# Autodesk Inventor assembly: ASY MSC 200 BACK
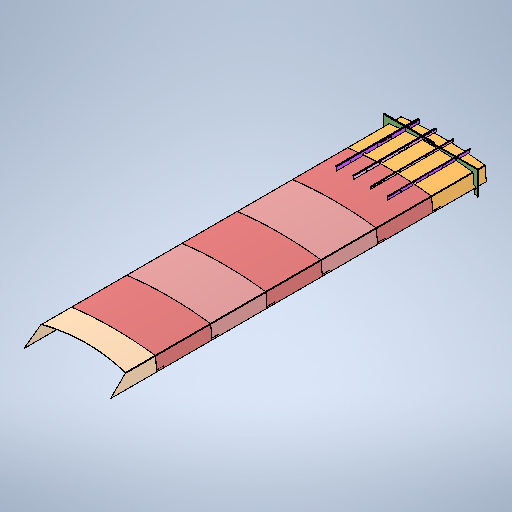
[picture p0: Inventor's stored thumbnail of the model, 512x512]
Saved by Autodesk Inventor 2025 (Build 290162010, 162A)
## iProperties
Created: 2024-07-19
Part Number: ASY MSC 200 BACK
Document SubType Name: Assembly
Designer: pokla
Stock Number: ASY МОО 200 спина
Mass: 379257 g
Surface Area: 351509 cm^2
Volume: 47407.1 cm^3
Density: 8 g/cm^3
Author: pokla
## Documents named in this file (10)
- C:\Users\admin\YandexDisk-badmisterfox\домашниий пк\Inventor\Manturovo\Manturovo_Se-clar\ASY MSC 200 BACK.iam
- C:\Users\admin\YandexDisk-badmisterfox\домашниий пк\Inventor\Manturovo\Manturovo_Se-clar\MSC 201 sheet back basic.ipt
- C:\Users\admin\YandexDisk-badmisterfox\домашниий пк\Inventor\Manturovo\Manturovo_Se-clar\MSC 203 rib back.ipt
- C:\Users\admin\YandexDisk-badmisterfox\домашниий пк\Inventor\Manturovo\Manturovo_Se-clar\MSC 202 BACK-neck.ipt
- C:\Users\admin\YandexDisk-badmisterfox\домашниий пк\Inventor\Manturovo\Manturovo_Se-clar\MSC 205 stringer back ^.ipt
- C:\Users\admin\YandexDisk-badmisterfox\домашниий пк\Inventor\Manturovo\Manturovo_Se-clar\MSC 206 stringer back ^^.ipt
- C:\Users\admin\YandexDisk-badmisterfox\домашниий пк\Inventor\Manturovo\Manturovo_Se-clar\MSC 208 sheet back mould.ipt
- C:\Users\admin\YandexDisk-badmisterfox\домашниий пк\Inventor\Manturovo\Manturovo_Se-clar\MSC 204 stringer back ^.ipt
- C:\Users\admin\YandexDisk-badmisterfox\домашниий пк\Inventor\Manturovo\Manturovo_Se-clar\MSC 207 stringer back ^^.ipt
- C:\Users\admin\YandexDisk-badmisterfox\домашниий пк\Inventor\Manturovo\Manturovo_Se-clar\MSC 208 sheet back START.ipt
## Components (74 placed, 9 different names)
1. MSC 201 sheet back basic.ipt:1 — Mate:1, Flush:2, Tangent:2, Rigid:65, Rigid:84, Mate:2, Mate:3, Flush:3
2. MSC 201 sheet back basic.ipt:2 — Rigid:65, Rigid:66
3. MSC 201 sheet back basic.ipt:3 — Rigid:66, Rigid:67
4. MSC 202 BACK-neck.ipt:1 — Rigid:69
5. MSC 201 sheet back basic.ipt:4 — Rigid:68, Rigid:69
6. MSC 201 sheet back basic.ipt:5 — Rigid:67, Rigid:68
7. MSC 205 stringer back ^.ipt:1 — Rigid:75, Rigid:76, Rigid:80
8. MSC 205 stringer back ^.ipt:2 — Rigid:77, Rigid:81
9. MSC 206 stringer back ^^.ipt:1 — Rigid:78, Rigid:82
10. MSC 206 stringer back ^^.ipt:2 — Rigid:79, Rigid:83
11. MSC 203 rib back.ipt:1 — Rigid:70, Rigid:73, Mate:3
12. MSC 203 rib back.ipt:2 — Rigid:70, Mate:2
13. MSC 204 stringer back ^.ipt:1 — Rigid:80
14. MSC 204 stringer back ^.ipt:2 — Rigid:81
15. MSC 207 stringer back ^^.ipt:1 — Rigid:82
16. MSC 207 stringer back ^^.ipt:2 — Rigid:83
17. MSC 208 sheet back START:1 — Rigid:84
18. MSC 208 sheet back mould.ipt:1 — Mate:1, Flush:2, Tangent:2, Rigid:22, Rigid:23
19. MSC 208 sheet back mould.ipt:2 — Rigid:22, Rigid:25
20. MSC 208 sheet back mould.ipt:3 — Rigid:23, Rigid:24
21. MSC 208 sheet back mould.ipt:4 — Rigid:24
22. MSC 208 sheet back mould.ipt:5 — Rigid:25, Rigid:27
23. MSC 208 sheet back mould.ipt:6 — Rigid:27
24. MSC 208 sheet back mould.ipt:7 — Rigid:31
25. MSC 208 sheet back mould.ipt:8 — Rigid:31
26. MSC 208 sheet back mould.ipt:9
27. MSC 208 sheet back mould.ipt:10
28. MSC 208 sheet back mould.ipt:11 — Rigid:33
29. MSC 208 sheet back mould.ipt:12 — Rigid:33
30. MSC 208 sheet back mould.ipt:13
31. MSC 203 rib back.ipt:3 — Rigid:73, Rigid:74, Rigid:78
32. MSC 203 rib back.ipt:4 — Rigid:74, Rigid:77, Rigid:79
33. MSC 203 rib back.ipt:5 — Rigid:75
34. MSC 203 rib back.ipt:6
35. MSC 203 rib back.ipt:7
36. MSC 203 rib back.ipt:8
37. MSC 203 rib back.ipt:9
38. MSC 203 rib back.ipt:10
39. MSC 203 rib back.ipt:11
40. MSC 203 rib back.ipt:12
41. MSC 203 rib back.ipt:13
42. MSC 203 rib back.ipt:14
43. MSC 203 rib back.ipt:15
44. MSC 203 rib back.ipt:16
45. MSC 203 rib back.ipt:17
46. MSC 203 rib back.ipt:18
47. MSC 203 rib back.ipt:19
48. MSC 203 rib back.ipt:20
49. MSC 203 rib back.ipt:21
50. MSC 203 rib back.ipt:22
51. MSC 203 rib back.ipt:23
52. MSC 203 rib back.ipt:24
53. MSC 203 rib back.ipt:25
54. MSC 203 rib back.ipt:26
55. MSC 206 stringer back ^^.ipt:3
56. MSC 205 stringer back ^.ipt:3 — Rigid:76
57. MSC 205 stringer back ^.ipt:4
58. MSC 206 stringer back ^^.ipt:4 — Flush:3
59. MSC 206 stringer back ^^.ipt:5
60. MSC 205 stringer back ^.ipt:5
61. MSC 205 stringer back ^.ipt:6
62. MSC 206 stringer back ^^.ipt:6
63. MSC 206 stringer back ^^.ipt:7
64. MSC 205 stringer back ^.ipt:7
65. MSC 205 stringer back ^.ipt:8
66. MSC 206 stringer back ^^.ipt:8
67. MSC 206 stringer back ^^.ipt:9
68. MSC 205 stringer back ^.ipt:9
69. MSC 205 stringer back ^.ipt:10
70. MSC 206 stringer back ^^.ipt:10
71. MSC 206 stringer back ^^.ipt:11
72. MSC 205 stringer back ^.ipt:11
73. MSC 205 stringer back ^.ipt:12
74. MSC 206 stringer back ^^.ipt:12
## Component patterns: (12 elements, first: MSC 203 rib back.ipt:3 + MSC 203 rib back.ipt:4), (5 elements, first: MSC 206 stringer back ^^.ipt:3 + MSC 205 stringer back ^.ipt:3 + MSC 205 stringer back ^.ipt:4 + MSC 206 stringer back ^^.ipt:4)
## Relationships (39: WeldJoint 33, Mate 3, Flush 2, Tangent 1)
- [WeldJoint]: MSC 205 stringer back ^.ipt:2 ↔ MSC 205 stringer back ^.ipt:4
- [WeldJoint]: MSC 206 stringer back ^^.ipt:1 ↔ MSC 206 stringer back ^^.ipt:3
- [WeldJoint]: MSC 206 stringer back ^^.ipt:2 ↔ MSC 206 stringer back ^^.ipt:4
- Mate:1: MSC 201 sheet back basic.ipt:1 ↔ MSC 208 sheet back mould.ipt:1
- Flush:2 (248.5 mm): MSC 201 sheet back basic.ipt:1 ↔ MSC 208 sheet back mould.ipt:1
- Tangent:2: MSC 201 sheet back basic.ipt:1 ↔ MSC 208 sheet back mould.ipt:1
- Rigid:22 [WeldJoint] (497 mm): MSC 208 sheet back mould.ipt:1 ↔ MSC 208 sheet back mould.ipt:2
- Rigid:23 [WeldJoint] (497 mm): MSC 208 sheet back mould.ipt:1 ↔ MSC 208 sheet back mould.ipt:3
- Rigid:24 [WeldJoint] (497 mm): MSC 208 sheet back mould.ipt:3 ↔ MSC 208 sheet back mould.ipt:4
- Rigid:25 [WeldJoint] (497 mm): MSC 208 sheet back mould.ipt:2 ↔ MSC 208 sheet back mould.ipt:5
- [WeldJoint] (497 mm): MSC 208 sheet back mould.ipt:6 ↔ MSC 208 sheet back mould.ipt:7
- Rigid:27 [WeldJoint] (497 mm): MSC 208 sheet back mould.ipt:5 ↔ MSC 208 sheet back mould.ipt:6
- [WeldJoint] (497 mm): MSC 208 sheet back mould.ipt:8 ↔ MSC 208 sheet back mould.ipt:9
- [WeldJoint] (497 mm): MSC 208 sheet back mould.ipt:10 ↔ MSC 208 sheet back mould.ipt:11
- [WeldJoint] (497 mm): MSC 208 sheet back mould.ipt:9 ↔ MSC 208 sheet back mould.ipt:10
- Rigid:31 [WeldJoint] (497 mm): MSC 208 sheet back mould.ipt:7 ↔ MSC 208 sheet back mould.ipt:8
- [WeldJoint] (497 mm): MSC 208 sheet back mould.ipt:12 ↔ MSC 208 sheet back mould.ipt:13
- Rigid:33 [WeldJoint] (497 mm): MSC 208 sheet back mould.ipt:11 ↔ MSC 208 sheet back mould.ipt:12
- Rigid:65 [WeldJoint]: MSC 201 sheet back basic.ipt:1 ↔ MSC 201 sheet back basic.ipt:2
- Rigid:66 [WeldJoint]: MSC 201 sheet back basic.ipt:2 ↔ MSC 201 sheet back basic.ipt:3
- Rigid:67 [WeldJoint]: MSC 201 sheet back basic.ipt:3 ↔ MSC 201 sheet back basic.ipt:5
- Rigid:68 [WeldJoint]: MSC 201 sheet back basic.ipt:4 ↔ MSC 201 sheet back basic.ipt:5
- Rigid:69 [WeldJoint]: MSC 202 BACK-neck.ipt:1 ↔ MSC 201 sheet back basic.ipt:4
- Rigid:70 [WeldJoint] (-100 mm): MSC 203 rib back.ipt:1 ↔ MSC 203 rib back.ipt:2
- Rigid:73 [WeldJoint] (-490 mm): MSC 203 rib back.ipt:1 ↔ MSC 203 rib back.ipt:3
- Rigid:74 [WeldJoint] (-100 mm): MSC 203 rib back.ipt:3 ↔ MSC 203 rib back.ipt:4
- Rigid:75 [WeldJoint] (2 mm): MSC 205 stringer back ^.ipt:1 ↔ MSC 203 rib back.ipt:5
- Rigid:76 [WeldJoint]: MSC 205 stringer back ^.ipt:1 ↔ MSC 205 stringer back ^.ipt:3
- Rigid:77 [WeldJoint] (2 mm): MSC 205 stringer back ^.ipt:2 ↔ MSC 203 rib back.ipt:4
- Rigid:78 [WeldJoint] (2 mm): MSC 206 stringer back ^^.ipt:1 ↔ MSC 203 rib back.ipt:3
- Rigid:79 [WeldJoint]: MSC 206 stringer back ^^.ipt:2 ↔ MSC 203 rib back.ipt:4
- Rigid:80 [WeldJoint]: MSC 205 stringer back ^.ipt:1 ↔ MSC 204 stringer back ^.ipt:1
- Rigid:81 [WeldJoint]: MSC 205 stringer back ^.ipt:2 ↔ MSC 204 stringer back ^.ipt:2
- Rigid:82 [WeldJoint]: MSC 206 stringer back ^^.ipt:1 ↔ MSC 207 stringer back ^^.ipt:1
- Rigid:83 [WeldJoint]: MSC 206 stringer back ^^.ipt:2 ↔ MSC 207 stringer back ^^.ipt:2
- Rigid:84 [WeldJoint]: MSC 201 sheet back basic.ipt:1 ↔ MSC 208 sheet back START:1
- Mate:2: MSC 201 sheet back basic.ipt:1 ↔ MSC 203 rib back.ipt:2
- Mate:3: MSC 201 sheet back basic.ipt:1 ↔ MSC 203 rib back.ipt:1
- Flush:3 (490 mm): MSC 201 sheet back basic.ipt:1 ↔ MSC 206 stringer back ^^.ipt:4
## Named parameters: d42_d41 = 497 mm, d44_d41 = 497 mm, d45_d42_d41 = 497 mm, d46_d43 = 497 mm, d48_d45_d42_d41 = 497 mm
